# Autodesk Inventor assembly: Busmodul Baugruppe
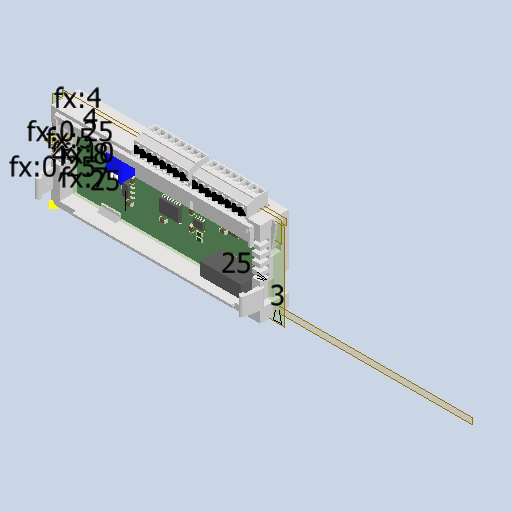
[picture p0: Inventor's stored thumbnail of the model, 512x512]
Saved by Autodesk Inventor 2025.2 (Build 292293000, 293)
## iProperties
Created: 2025-11-01
Part Number: Busmodul Baugruppe
Document SubType Name: Assembly
Designer: leowa
Author: leowa
## Documents named in this file (5)
- C:\Users\leowa\OneDrive - Fachhochschule Aachen\FH\8. Semester\CAN Tram CAD\Module\Busmodul Baugruppe.iam
- C:\Users\leowa\OneDrive - Fachhochschule Aachen\FH\8. Semester\CAN Tram CAD\Gehäuse\Generisches Gehäuse V2.ipt
- C:\Users\leowa\OneDrive - Fachhochschule Aachen\FH\8. Semester\CAN Tram CAD\Kaufteile\Terminalstecker 8fach\0395000008.iam
- C:\Users\leowa\OneDrive - Fachhochschule Aachen\FH\8. Semester\CAN Tram CAD\Gehäuse\Busmodul Gehäuse Deckel.ipt
- C:\Users\leowa\OneDrive - Fachhochschule Aachen\FH\8. Semester\CAN Tram CAD\Platinen\Busmodul\Busmodul\Busmodul.iam
## Components (5 placed, 4 different names)
1. Generisches Gehäuse V2:1 — Passend:1, Passend:2, Passend:3, Fluchtend:1, Fluchtend:2, Passend:4
2. 0395000008:1 [sub-assembly] — Passend:5, Passend:6
3. Busmodul Gehäuse Deckel:1 — Fluchtend:1, Fluchtend:2, Passend:4
4. Busmodul:1 [sub-assembly] — Passend:1, Passend:2, Passend:3, Passend:5, Passend:6, Passend:7, Passend:8
5. 0395000008:2 [sub-assembly] — Passend:7, Passend:8
## Relationships (10: Mate 8, Flush 2)
- Passend:1 [Mate]: Generisches Gehäuse V2:1 ↔ Busmodul:1
- Passend:2 [Mate]: Generisches Gehäuse V2:1 ↔ Busmodul:1
- Passend:3 [Mate] (1 mm): Generisches Gehäuse V2:1 ↔ Busmodul:1
- Fluchtend:1 [Flush]: Generisches Gehäuse V2:1 ↔ Busmodul Gehäuse Deckel:1
- Fluchtend:2 [Flush]: Generisches Gehäuse V2:1 ↔ Busmodul Gehäuse Deckel:1
- Passend:4 [Mate]: Generisches Gehäuse V2:1 ↔ Busmodul Gehäuse Deckel:1
- Passend:5 [Mate]: 0395000008:1 ↔ Busmodul:1
- Passend:6 [Mate]: 0395000008:1 ↔ Busmodul:1
- Passend:7 [Mate]: Busmodul:1 ↔ 0395000008:2
- Passend:8 [Mate]: Busmodul:1 ↔ 0395000008:2
